# Autodesk Inventor assembly: Drive
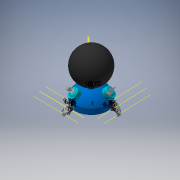
[picture p0: Inventor's stored thumbnail of the model, 180x180]
Saved by Autodesk Inventor 2018.3 (Build 223284000, 284)
## iProperties
Created: 2018-06-30
Part Number: Drive
Material: Generisch
Document SubType Name: Assembly
Designer: JochenAlt
Author: JochenAlt
## Documents named in this file (5)
- D:\Projects\FlowerPot\CAD\Drive.iam
- D:\Projects\FlowerPot\CAD\DriveChain.iam
- D:\Projects\FlowerPot\CAD\Sphere.ipt
- D:\Projects\FlowerPot\CAD\Spindle\SpindleThread.ipt
- D:\Projects\FlowerPot\CAD\Form.iam
## Components (8 placed, 4 different names)
1. DriveChain:1 [sub-assembly] — Passend:48, Passend:49, Passend:50, Passend:51, Passend:54, Passend:55
2. DriveChain:2 [sub-assembly] — Passend:47, Passend:49, Passend:50, Passend:53, Passend:57, Passend:58
3. DriveChain:3 [sub-assembly] — Passend:26, Passend:27, Tangential:1, Passend:47, Passend:48, Passend:51, Passend:52, Passend:56, Tangential:2
4. Sphere:1 — Tangential:1, Passend:38, Tangential:2
5. SpindleThread:1 — Passend:26, Passend:27, Passend:39, Passend:52, Passend:56
6. SpindleThread:2 — Passend:54, Passend:55
7. SpindleThread:3 — Passend:40, Passend:53, Passend:57
8. Form:1 [sub-assembly] — Passend:39, Passend:40
## Relationships (19: Mate 17, Tangent 2)
- Passend:26 [Mate]: DriveChain:3 ↔ SpindleThread:1
- Passend:27 [Mate]: DriveChain:3 ↔ SpindleThread:1
- Tangential:1: DriveChain:3 ↔ Sphere:1
- Passend:38 [Mate]: Sphere:1
- Passend:39 [Mate]: SpindleThread:1 ↔ Form:1
- Passend:40 [Mate]: SpindleThread:3 ↔ Form:1
- Passend:47 [Mate]: DriveChain:2 ↔ DriveChain:3
- Passend:48 [Mate]: DriveChain:1 ↔ DriveChain:3
- Passend:49 [Mate]: DriveChain:1 ↔ DriveChain:2
- Passend:50 [Mate]: DriveChain:1 ↔ DriveChain:2
- Passend:51 [Mate]: DriveChain:1 ↔ DriveChain:3
- Passend:52 [Mate]: DriveChain:3 ↔ SpindleThread:1
- Passend:53 [Mate]: DriveChain:2 ↔ SpindleThread:3
- Passend:54 [Mate]: DriveChain:1 ↔ SpindleThread:2
- Passend:55 [Mate]: DriveChain:1 ↔ SpindleThread:2
- Passend:56 [Mate]: DriveChain:3 ↔ SpindleThread:1
- Passend:57 [Mate]: DriveChain:2 ↔ SpindleThread:3
- Passend:58 [Mate]: DriveChain:2
- Tangential:2: DriveChain:3 ↔ Sphere:1
